# Autodesk Inventor assembly: assemblyxrail
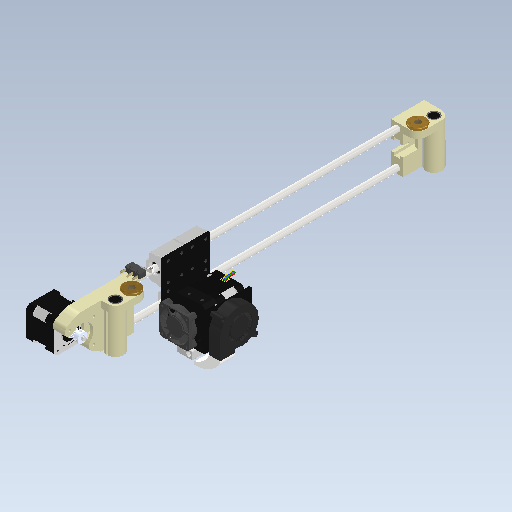
[picture p0: Inventor's stored thumbnail of the model, 512x512]
Saved by Autodesk Inventor 2020.2 (Build 242310000, 310)
## iProperties
Created: 2020-07-30
Part Number: assemblyxrail
Document SubType Name: Assembly
Designer: JK
Author: JK
## Documents named in this file (20)
- C:\Users\JK\Documents\Inventor\Anet Upgrade\assemblyxrail.iam
- C:\Users\JK\Documents\Inventor\Anet Upgrade\xaxissupport1.ipt
- C:\Users\JK\Documents\Inventor\Anet Upgrade\xaxissupport2.ipt
- C:\Users\JK\Documents\Inventor\Anet Upgrade\8x435axis.ipt
- C:\Users\JK\Documents\Inventor\Anet Upgrade\MOTOR.ipt
- C:\Users\JK\Documents\Inventor\Anet Upgrade\gantry.ipt
- C:\Users\JK\Documents\Inventor\Anet Upgrade\LinearBearing8mm.iam
- C:\Users\JK\Documents\Inventor\Anet Upgrade\LM8UU 8mm Linear Bearing.ipt
- C:\Users\JK\Documents\Inventor\Anet Upgrade\ACMENut.ipt
- C:\Users\JK\Documents\Inventor\Anet Upgrade\HotBlock.ipt
- C:\Users\JK\Documents\Inventor\Anet Upgrade\nozzle.ipt
- C:\Users\JK\Documents\Inventor\Anet Upgrade\Fan40x40.ipt
- C:\Users\JK\Documents\Inventor\Anet Upgrade\throat.ipt
- C:\Users\JK\Documents\Inventor\Anet Upgrade\HeatSink.ipt
- C:\Users\JK\Documents\Inventor\Anet Upgrade\EndStop.ipt
- C:\Users\JK\Documents\Inventor\Anet Upgrade\GT2-16pulley.iam
- C:\Users\JK\Documents\Inventor\Anet Upgrade\ExtuderPartA.ipt
- C:\Users\JK\Documents\Inventor\Anet Upgrade\ExtruderPartB.ipt
- C:\Users\JK\Documents\Inventor\Anet Upgrade\Radial-Cooling-Fan-5015-DC12V.iam
- C:\Users\JK\Documents\Inventor\Anet Upgrade\Duct.ipt
## Components (27 placed, 19 different names)
1. xaxissupport1:1 — Mate:19, Mate:20, Flush:5, Flush:6, Mate:23, Mate:24
2. xaxissupport2:1 — Mate:17, Mate:18, Flush:3, Flush:4, Mate:21, Mate:22, Mate:41, Mate:42, Angle:6, Flush:7
3. Wał:1
4. Wał:2
5. MOTOR:1 — Mate:43
6. gantry:1 — Mate:25, Angle:3, Mate:40, Mate:47, Mate:48, Angle:7, Mate:51, Mate:52, Mate:53
7. LinearBearing8mm:1 [sub-assembly]
8. LinearBearing8mm:2 [sub-assembly]
9. LinearBearing8mm:3 [sub-assembly]
10. LM8UU 8mm Linear Bearing:1 — Mate:18, Flush:3
11. LM8UU 8mm Linear Bearing:2 — Mate:17, Flush:4
12. LM8UU 8mm Linear Bearing:3 — Mate:20, Flush:6
13. LM8UU 8mm Linear Bearing:4 — Mate:19, Flush:5
14. ACMENut:1 — Mate:21, Mate:22
15. ACMENut:2 — Mate:23, Mate:24
16. MOTOR:2 — Mate:34, Angle:4, Angle:5, Mate:45, Mate:46, Mate:49, Angle:7
17. HotBlock:1 — Mate:25, Mate:26, Mate:27, Mate:31, Angle:4, Mate:40
18. nozzle:1 — Mate:26, Mate:27, Mate:32
19. 40_wentylator 40mm:1 — Mate:34, Angle:3, Mate:38, Mate:39
20. throat:1 — Mate:31, Mate:32, Mate:44
21. 36_radiator:1 — Mate:38, Mate:39, Angle:5, Mate:50
22. 25T0397-001:1 — Mate:41, Mate:42, Angle:6
23. GT2-16pulley:1 [sub-assembly] — Mate:43, Flush:7
24. ExtuderPartA:1 — Mate:44, Mate:47, Mate:48, Mate:49, Flush:8, Mate:50
25. ExtruderPartB:1 — Mate:45, Mate:46, Flush:8
26. Radial-Cooling-Fan-5015-DC12V:1 [sub-assembly] — Mate:51, Mate:52, Mate:53, Mate:54, Mate:55, Mate:56
27. Duct:1 — Mate:54, Mate:55, Mate:56
## Relationships (64: Mate 49, Flush 8, Angle 7)
- [Mate]: xaxissupport1:1 ↔ xaxissupport2:1
- [Mate]: xaxissupport1:1 ↔ xaxissupport2:1
- [Mate]: xaxissupport1:1 ↔ Wał:2
- [Mate]: xaxissupport1:1 ↔ Wał:1
- [Flush]: Wał:1 ↔ Wał:2
- [Mate]: xaxissupport2:1 ↔ MOTOR:1
- [Mate]: xaxissupport2:1 ↔ MOTOR:1
- [Angle] (0 deg): xaxissupport2:1 ↔ MOTOR:1
- [Mate] (-32 mm): xaxissupport2:1 ↔ Wał:2
- [Flush]: xaxissupport1:1 ↔ Wał:2
- [Mate]: gantry:1 ↔ LinearBearing8mm:1
- [Mate]: gantry:1 ↔ LinearBearing8mm:1
- [Mate]: gantry:1 ↔ LinearBearing8mm:1
- [Mate]: LinearBearing8mm:1 ↔ LinearBearing8mm:2
- [Mate]: gantry:1 ↔ LinearBearing8mm:2
- [Mate]: gantry:1 ↔ LinearBearing8mm:3
- [Mate]: gantry:1 ↔ LinearBearing8mm:3
- [Angle] (0 deg): LinearBearing8mm:2 ↔ LinearBearing8mm:3
- [Mate]: Wał:1 ↔ LinearBearing8mm:3
- [Mate]: Wał:2 ↔ LinearBearing8mm:2
- Mate:17: xaxissupport2:1 ↔ LM8UU 8mm Linear Bearing:2
- Mate:18: xaxissupport2:1 ↔ LM8UU 8mm Linear Bearing:1
- Flush:3: xaxissupport2:1 ↔ LM8UU 8mm Linear Bearing:1
- Flush:4: xaxissupport2:1 ↔ LM8UU 8mm Linear Bearing:2
- Mate:19: xaxissupport1:1 ↔ LM8UU 8mm Linear Bearing:4
- Mate:20: xaxissupport1:1 ↔ LM8UU 8mm Linear Bearing:3
- Flush:5: xaxissupport1:1 ↔ LM8UU 8mm Linear Bearing:4
- Flush:6: xaxissupport1:1 ↔ LM8UU 8mm Linear Bearing:3
- Mate:21: xaxissupport2:1 ↔ ACMENut:1
- Mate:22: xaxissupport2:1 ↔ ACMENut:1
- Mate:23: xaxissupport1:1 ↔ ACMENut:2
- Mate:24: xaxissupport1:1 ↔ ACMENut:2
- Mate:25: gantry:1 ↔ HotBlock:1
- Mate:26: HotBlock:1 ↔ nozzle:1
- Mate:27 (2 mm): HotBlock:1 ↔ nozzle:1
- Mate:31: HotBlock:1 ↔ throat:1
- Mate:32: nozzle:1 ↔ throat:1
- Mate:34: MOTOR:2 ↔ 40_wentylator 40mm:1
- Angle:3 (0 deg): gantry:1 ↔ 40_wentylator 40mm:1
- Mate:38: 40_wentylator 40mm:1 ↔ 36_radiator:1
- Mate:39: 40_wentylator 40mm:1 ↔ 36_radiator:1
- Angle:4 (0 deg): MOTOR:2 ↔ HotBlock:1
- Mate:40 (10 mm): gantry:1 ↔ HotBlock:1
- Angle:5 (0 deg): MOTOR:2 ↔ 36_radiator:1
- Mate:41: xaxissupport2:1 ↔ 25T0397-001:1
- Mate:42: xaxissupport2:1 ↔ 25T0397-001:1
- Angle:6 (0 deg): xaxissupport2:1 ↔ 25T0397-001:1
- Mate:43: MOTOR:1 ↔ GT2-16pulley:1
- Flush:7 (-0.5 mm): xaxissupport2:1 ↔ GT2-16pulley:1
- Mate:44: throat:1 ↔ ExtuderPartA:1
- Mate:45: MOTOR:2 ↔ ExtruderPartB:1
- Mate:46: MOTOR:2 ↔ ExtruderPartB:1
- Mate:47: gantry:1 ↔ ExtuderPartA:1
- Mate:48: gantry:1 ↔ ExtuderPartA:1
- Mate:49: MOTOR:2 ↔ ExtuderPartA:1
- Flush:8: ExtuderPartA:1 ↔ ExtruderPartB:1
- Mate:50: 36_radiator:1 ↔ ExtuderPartA:1
- Angle:7 (0 deg): gantry:1 ↔ MOTOR:2
- Mate:51: gantry:1 ↔ Radial-Cooling-Fan-5015-DC12V:1
- Mate:52: gantry:1 ↔ Radial-Cooling-Fan-5015-DC12V:1
- Mate:53: gantry:1 ↔ Radial-Cooling-Fan-5015-DC12V:1
- Mate:54: Radial-Cooling-Fan-5015-DC12V:1 ↔ Duct:1
- Mate:55: Radial-Cooling-Fan-5015-DC12V:1 ↔ Duct:1
- Mate:56: Radial-Cooling-Fan-5015-DC12V:1 ↔ Duct:1
## Named parameters: d0_d17 = 0 deg, d1_d18 = 0 mm, d2_d19 = 0 mm
